# Autodesk Inventor assembly: GearboxAssembly
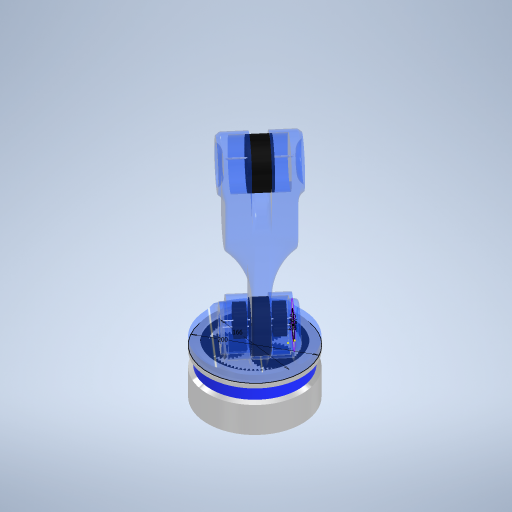
[picture p0: Inventor's stored thumbnail of the model, 512x512]
Saved by Autodesk Inventor 2024 (Build 280153000, 153)
## iProperties
Created: 2023-07-07
Part Number: GearboxAssembly
Document SubType Name: Assembly
Designer: westy
Author: westy
## Documents named in this file (18)
- D:\Autodesk\RoboticArmparts\GearboxAssembly.iam
- D:\Autodesk\RoboticArmparts\PlanetarygearboxBase.ipt
- D:\Autodesk\RoboticArmparts\GearboxAssembly\Design Accelerator\Spur Gears15.iam
- D:\Autodesk\RoboticArmparts\GearboxAssembly\Design Accelerator\Spur Gears3.iam
- D:\Autodesk\RoboticArmparts\Base.ipt
- D:\Autodesk\RoboticArmparts\GearboxAssembly\Design Accelerator\Spur Gears5.iam
- D:\Autodesk\RoboticArmparts\GearboxAssembly\Design Accelerator\Spur Gears6.iam
- D:\Autodesk\RoboticArmparts\ArmBase.ipt
- D:\Autodesk\RoboticArmparts\Shaft.ipt
- D:\Autodesk\RoboticArmparts\GearboxAssembly\Design Accelerator\Spur Gears13.iam
- D:\Autodesk\RoboticArmparts\GearboxAssembly\Design Accelerator\Spur Gears21.iam
- D:\Autodesk\RoboticArmparts\GearboxAssembly\Design Accelerator\Spur Gears17.iam
- D:\Autodesk\RoboticArmparts\GearboxAssembly\Design Accelerator\Spur Gears26.iam
- D:\Autodesk\RoboticArmparts\GearboxAssembly\Design Accelerator\Spur Gears27.iam
- D:\Autodesk\RoboticArmparts\ArmPiece2.ipt
- D:\Autodesk\RoboticArmparts\Shaft2.ipt
- D:\Autodesk\RoboticArmparts\GearboxAssembly\Design Accelerator\Spur Gears23.iam
- D:\Autodesk\RoboticArmparts\GearboxAssembly\Design Accelerator\Spur Gears24.iam
## Components (21 placed, 7 different names)
1. PlanetarygearboxBase:1 — Mate:1, Mate:2, Mate:7, Rotation:5, Mate:8, Mate:9, Rotation:6, Mate:10
2. Spur Gears:2 [sub-assembly]
3. Spur Gears:3 [sub-assembly] — Mate:7, Rotation:4, Rotation:5, Flush:4, Mate:8
4. Base:2 — Mate:1, Mate:2, Mate:3, Mate:4, Mate:5, Mate:6
5. Spur Gears:4 [sub-assembly] — Mate:6, Rotation:2, Flush:2
6. Spur Gears:5 [sub-assembly] — Mate:4, Rotation:3, Flush:3, Rotation:4, Flush:4
7. Spur Gears:6 [sub-assembly] — Mate:5, Rotation:1, Flush:1
8. Spur Gears:7 [sub-assembly] — Mate:3, Rotation:1, Flush:1, Rotation:2, Flush:2, Rotation:3, Flush:3
9. ArmBase:1 — Mate:9, Rotation:6, Mate:10, Mate:11, Mate:12, Mate:13, Mate:14, Mate:17, Mate:27
10. Shaft:1 — Mate:12, Mate:14, Mate:18, Mate:21, Rotation:8
11. Shaft:2 — Mate:11, Mate:13, Mate:19, Mate:20, Rotation:7, Rotation:9, Flush:5, Flush:6, Mate:22, Rotation:10, Mate:24, Mate:25
12. Spur Gears:10 [sub-assembly]
13. Spur Gears:16 [sub-assembly] — Mate:20, Mate:21, Rotation:7, Rotation:8, Flush:6
14. Spur Gears:17 [sub-assembly] — Mate:17, Mate:22, Rotation:11, Mate:26, Rotation:12
15. Spur Gears:18 [sub-assembly] — Mate:18, Mate:19, Rotation:9, Flush:5
16. Spur Gears:19 [sub-assembly] — Rotation:10, Mate:24, Mate:25, Rotation:11
17. ArmPiece2:1 — Mate:26, Rotation:12, Mate:27, Mate:28, Flush:7, Mate:29, Flush:8, Mate:32, Mate:33, Flush:9
18. Shaft2:1 — Mate:28, Flush:7, Mate:31
19. Shaft2:2 — Mate:29, Flush:8, Mate:30
20. Spur Gears:22 [sub-assembly] — Mate:30, Mate:31, Mate:32, Rotation:13
21. Spur Gears:23 [sub-assembly] — Rotation:13, Mate:33, Flush:9
## Relationships (52: Mate 30, RelateRotation 13, Flush 9)
- Mate:1: PlanetarygearboxBase:1 ↔ Base:2
- Mate:2: PlanetarygearboxBase:1 ↔ Base:2
- Mate:3: Base:2 ↔ Spur Gears:7
- Mate:4: Base:2 ↔ Spur Gears:5
- Mate:5: Base:2 ↔ Spur Gears:6
- Mate:6: Base:2 ↔ Spur Gears:4
- Mate:7: PlanetarygearboxBase:1 ↔ Spur Gears:3
- Rotation:1 [RelateRotation] (0.3333 ul): Spur Gears:6 ↔ Spur Gears:7
- Flush:1: Spur Gears:6 ↔ Spur Gears:7
- Rotation:2 [RelateRotation] (3 ul): Spur Gears:4 ↔ Spur Gears:7
- Flush:2: Spur Gears:4 ↔ Spur Gears:7
- Rotation:3 [RelateRotation] (3 ul): Spur Gears:5 ↔ Spur Gears:7
- Flush:3: Spur Gears:5 ↔ Spur Gears:7
- Rotation:4 [RelateRotation] (2.4 ul): Spur Gears:3 ↔ Spur Gears:5
- Rotation:5 [RelateRotation] (1 ul): PlanetarygearboxBase:1 ↔ Spur Gears:3
- Flush:4: Spur Gears:3 ↔ Spur Gears:5
- Mate:8: PlanetarygearboxBase:1 ↔ Spur Gears:3
- Mate:9: PlanetarygearboxBase:1 ↔ ArmBase:1
- Rotation:6 [RelateRotation] (1 ul): PlanetarygearboxBase:1 ↔ ArmBase:1
- Mate:10: PlanetarygearboxBase:1 ↔ ArmBase:1
- Mate:11: ArmBase:1 ↔ Shaft:2
- Mate:12: ArmBase:1 ↔ Shaft:1
- Mate:13: ArmBase:1 ↔ Shaft:2
- Mate:14: ArmBase:1 ↔ Shaft:1
- Mate:17: ArmBase:1 ↔ Spur Gears:17
- Mate:18: Shaft:1 ↔ Spur Gears:18
- Mate:19: Shaft:2 ↔ Spur Gears:18
- Mate:20: Shaft:2 ↔ Spur Gears:16
- Mate:21: Shaft:1 ↔ Spur Gears:16
- Rotation:7 [RelateRotation] (1 ul): Shaft:2 ↔ Spur Gears:16
- Rotation:8 [RelateRotation] (1 ul): Shaft:1 ↔ Spur Gears:16
- Rotation:9 [RelateRotation] (1 ul): Shaft:2 ↔ Spur Gears:18
- Flush:5 (15 mm): Shaft:2 ↔ Spur Gears:18
- Flush:6 (15 mm): Shaft:2 ↔ Spur Gears:16
- Mate:22 (40 mm): Shaft:2 ↔ Spur Gears:17
- Rotation:10 [RelateRotation] (1 ul): Shaft:2 ↔ Spur Gears:19
- Mate:24 (-70 mm): Shaft:2 ↔ Spur Gears:19
- Mate:25: Shaft:2 ↔ Spur Gears:19
- Rotation:11 [RelateRotation] (0.66 ul): Spur Gears:17 ↔ Spur Gears:19
- Mate:26: Spur Gears:17 ↔ ArmPiece2:1
- Rotation:12 [RelateRotation] (1 ul): Spur Gears:17 ↔ ArmPiece2:1
- Mate:27: ArmBase:1 ↔ ArmPiece2:1
- Mate:28: ArmPiece2:1 ↔ Shaft2:1
- Flush:7 (5 mm): ArmPiece2:1 ↔ Shaft2:1
- Mate:29: ArmPiece2:1 ↔ Shaft2:2
- Flush:8 (5 mm): ArmPiece2:1 ↔ Shaft2:2
- Mate:30: Shaft2:2 ↔ Spur Gears:22
- Mate:31: Shaft2:1 ↔ Spur Gears:22
- Mate:32 (-5 mm): ArmPiece2:1 ↔ Spur Gears:22
- Rotation:13 [RelateRotation] (1 ul): Spur Gears:22 ↔ Spur Gears:23
- Mate:33: ArmPiece2:1 ↔ Spur Gears:23
- Flush:9 (-35 mm): ArmPiece2:1 ↔ Spur Gears:23
